# Autodesk Inventor assembly: Alice._newiam
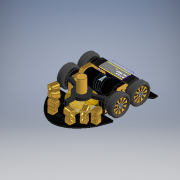
[picture p0: Inventor's stored thumbnail of the model, 180x180]
Saved by Autodesk Inventor 2016 (Build 200138000, 138)
## iProperties
Created: 2017-06-11
Part Number: Alice._newiam
Material: 一般
Document SubType Name: Assembly
Designer: kota
Author: kota
## Documents named in this file (7)
- C:\Users\B4_Ohno\Dropbox\AliCe\MicroMouse2016\Alice._new.iam
- C:\Users\B4_Ohno\Dropbox\AliCe\MicroMouse2016\shitaita_new.ipt
- C:\Users\B4_Ohno\Dropbox\AliCe\MicroMouse2016\LED_mount.ipt
- C:\Users\B4_Ohno\Dropbox\AliCe\MicroMouse2016\Assembly1.iam
- C:\Users\B4_Ohno\Dropbox\AliCe\MicroMouse2016\LCD.iam
- C:\Users\B4_Ohno\Dropbox\AliCe\MicroMouse2016\AliCe_Motor_l.iam
- C:\Users\B4_Ohno\Dropbox\AliCe\MicroMouse2016\AliCe_Motor_R.iam
## Components (11 placed, 6 different names)
1. shitaita_new:1 — メイト:1, メイト:2, メイト:3, メイト:4, メイト:5, メイト:6, メイト:7, メイト:8, メイト:9, メイト:12, メイト:13, メイト:14, メイト:15, メイト:16, メイト:17, メイト:18, メイト:19, メイト:20, メイト:21, メイト:22, フラッシュ:1, フラッシュ:2, リジッド:1, リジッド:2
2. LED_mount:1 — メイト:1, メイト:2, メイト:3
3. LED_mount:2 — メイト:4, メイト:5, メイト:6
4. LED_mount:3 — メイト:7, メイト:8, メイト:9
5. LED_mount:4 — メイト:12, メイト:13, メイト:14
6. LED_mount:5 — メイト:15, メイト:16, メイト:17
7. LED_mount:6 — メイト:18, メイト:19, メイト:20
8. LCD:1 [sub-assembly] — メイト:24, フラッシュ:3, フラッシュ:4
9. Assembly1:1 [sub-assembly] — メイト:21, メイト:22, フラッシュ:1, フラッシュ:2, メイト:23
10. AliCe_Motor_l:1 [sub-assembly] — リジッド:1, フラッシュ:3, フラッシュ:4
11. AliCe_Motor_R:1 [sub-assembly] — リジッド:2, メイト:23, メイト:24
## Relationships (28: Mate 22, Flush 4, WeldJoint 2)
- メイト:1 [Mate]: shitaita_new:1 ↔ LED_mount:1
- メイト:2 [Mate]: shitaita_new:1 ↔ LED_mount:1
- メイト:3 [Mate]: shitaita_new:1 ↔ LED_mount:1
- メイト:4 [Mate]: shitaita_new:1 ↔ LED_mount:2
- メイト:5 [Mate]: shitaita_new:1 ↔ LED_mount:2
- メイト:6 [Mate]: shitaita_new:1 ↔ LED_mount:2
- メイト:7 [Mate]: shitaita_new:1 ↔ LED_mount:3
- メイト:8 [Mate]: shitaita_new:1 ↔ LED_mount:3
- メイト:9 [Mate]: shitaita_new:1 ↔ LED_mount:3
- メイト:12 [Mate]: shitaita_new:1 ↔ LED_mount:4
- メイト:13 [Mate]: shitaita_new:1 ↔ LED_mount:4
- メイト:14 [Mate]: shitaita_new:1 ↔ LED_mount:4
- メイト:15 [Mate]: shitaita_new:1 ↔ LED_mount:5
- メイト:16 [Mate]: shitaita_new:1 ↔ LED_mount:5
- メイト:17 [Mate]: shitaita_new:1 ↔ LED_mount:5
- メイト:18 [Mate]: shitaita_new:1 ↔ LED_mount:6
- メイト:19 [Mate]: shitaita_new:1 ↔ LED_mount:6
- メイト:20 [Mate]: shitaita_new:1 ↔ LED_mount:6
- メイト:21 [Mate]: shitaita_new:1 ↔ Assembly1:1
- メイト:22 [Mate]: shitaita_new:1 ↔ Assembly1:1
- フラッシュ:1 [Flush]: shitaita_new:1 ↔ Assembly1:1
- フラッシュ:2 [Flush]: shitaita_new:1 ↔ Assembly1:1
- リジッド:1 [WeldJoint]: shitaita_new:1 ↔ AliCe_Motor_l:1
- リジッド:2 [WeldJoint]: shitaita_new:1 ↔ AliCe_Motor_R:1
- メイト:23 [Mate]: Assembly1:1 ↔ AliCe_Motor_R:1
- メイト:24 [Mate]: LCD:1 ↔ AliCe_Motor_R:1
- フラッシュ:3 [Flush]: LCD:1 ↔ AliCe_Motor_l:1
- フラッシュ:4 [Flush]: LCD:1 ↔ AliCe_Motor_l:1
